# Autodesk Inventor assembly: HM1-1002_CAM1
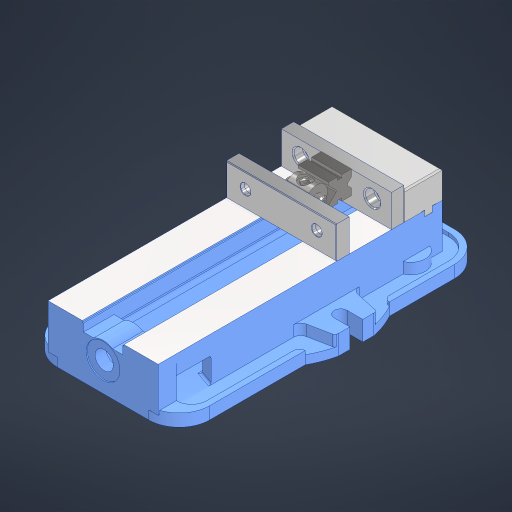
[picture p0: Inventor's stored thumbnail of the model, 512x512]
Saved by Autodesk Inventor 2024.3 (Build 283343000, 343)
## iProperties
Created: 2024-06-04
Part Number: HM1-1002_CAM1
Document SubType Name: Assembly
Designer: fablabadmin
Author: fablabadmin
## Documents named in this file (7)
- C:\Users\fablabadmin\Documents\_Benjamin_S\_3dCAD\HHVerkstad\Hammer\_CAM\HM1-1002_CAM1.iam
- C:\Users\fablabadmin\Documents\_Benjamin_S\_3dCAD\_Config\KemmlerVise\OP1-KemmlerVise.iam
- C:\Users\fablabadmin\Documents\Inventor\Content Center Files\R2024\en-US\StandardJaw\JawSTD-Aluminum 6061.ipt
- C:\Users\fablabadmin\Documents\_Benjamin_S\_3dCAD\HHVerkstad\Hammer\HM1-1002.ipt
- C:\Users\fablabadmin\Documents\Inventor\Content Center Files\R2024\en-US\V-Block\vBlock.ipt
- C:\Users\fablabadmin\Documents\_Benjamin_S\_3dCAD\HHVerkstad\Hammer\_CAM\OP1_Stock.ipt
- C:\Users\fablabadmin\Documents\_Benjamin_S\_3dCAD\_Config\_CAM_SIM\FixtureParts\parallels3mm.xlsx
## Components (6 placed, 5 different names)
1. HM1-1002:1 — Mate:6, Flush:5, Flush:6, Angle:1
2. OP1_Stock:1 — Mate:6, Flush:5, Flush:6, Tangent:1, Tangent:2, Tangent:3
3. OP1-KemmlerVise:1 [sub-assembly] — Mate:1, Mate:2, Flush:1, Mate:3, Flush:3, Mate:5
4. V-Block vBlock:1 — Flush:4, Mate:4, Mate:5, Tangent:1, Tangent:2, Angle:1
5. StandardJaw JawSTD-Aluminum 6061:1 — Mate:1, Flush:1, Flush:2, Mate:3, Mate:4
6. StandardJaw JawSTD-Aluminum 6061:2 — Mate:2, Flush:2, Tangent:3
## Relationships (16: Mate 6, Flush 6, Tangent 3, Angle 1)
- Mate:1: OP1-KemmlerVise:1 ↔ StandardJaw JawSTD-Aluminum 6061:1
- Mate:2: OP1-KemmlerVise:1 ↔ StandardJaw JawSTD-Aluminum 6061:2
- Flush:1: OP1-KemmlerVise:1 ↔ StandardJaw JawSTD-Aluminum 6061:1
- Flush:2: StandardJaw JawSTD-Aluminum 6061:1 ↔ StandardJaw JawSTD-Aluminum 6061:2
- Mate:3: OP1-KemmlerVise:1 ↔ StandardJaw JawSTD-Aluminum 6061:1
- Flush:3: OP1-KemmlerVise:1
- Flush:4: V-Block vBlock:1
- Mate:4: V-Block vBlock:1 ↔ StandardJaw JawSTD-Aluminum 6061:1
- Mate:5 (13 mm): OP1-KemmlerVise:1 ↔ V-Block vBlock:1
- Mate:6: HM1-1002:1 ↔ OP1_Stock:1
- Flush:5: HM1-1002:1 ↔ OP1_Stock:1
- Flush:6: HM1-1002:1 ↔ OP1_Stock:1
- Tangent:1: OP1_Stock:1 ↔ V-Block vBlock:1
- Tangent:2: OP1_Stock:1 ↔ V-Block vBlock:1
- Angle:1 (0 deg): HM1-1002:1 ↔ V-Block vBlock:1
- Tangent:3: OP1_Stock:1 ↔ StandardJaw JawSTD-Aluminum 6061:2
## Named parameters: PRL13 = 13 mm, PRL16 = 16 mm, PRL19 = 19 mm, PRL22 = 22 mm, PRL28 = 28 mm, PRL31 = 31 mm, PRL35 = 35 mm, PRL38 = 38 mm, PRL41 = 41 mm
